# Autodesk Inventor assembly: RobotConceptTesting
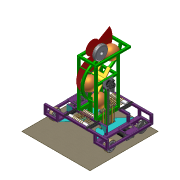
[picture p0: Inventor's stored thumbnail of the model, 180x180]
Saved by Autodesk Inventor 2012 (Build 160160000, 160)
## iProperties
Created: 2012-01-09
Part Number: RobotConceptTesting
Document SubType Name: Assembly
Designer: JesseK
Mass: 20586.5 g
Surface Area: 79739.9 cm^2
Volume: 10731.8 cm^3
Density: 1.91828 g/cm^3
Author: JesseK
## Documents named in this file (8)
- Z:\UserData\Documents\Inventor\team1885frc\Robot2012\RobotConceptTesting.iam
- Z:\UserData\Documents\Inventor\team1885frc\Robot2012\DriveTrain\DiveTrain_FullAssembly.iam
- Z:\UserData\Documents\Inventor\team1885frc\Robot2012\Concepts\Floor.ipt
- Z:\UserData\Documents\Inventor\team1885frc\Robot2012\Conveyor2\ConveyorFullAssembly.iam
- Z:\UserData\Documents\Inventor\team1885frc\Robot2012\Concepts\ShooterSketch.ipt
- Z:\UserData\Documents\Inventor\team1885frc\Robot2012\Conveyor2\Conveyor_Roller_Cross.ipt
- Z:\UserData\Documents\Inventor\team1885frc\Robot2012\Conveyor2\PitchingArmConcept.ipt
- Z:\UserData\Documents\Inventor\team1885frc\Field\Compressed ball.ipt
## Components (10 placed, 7 different names)
1. DiveTrain_FullAssembly:1 [sub-assembly] — Tangent:1, Flush:1, Flush:2, Flush:5, Mate:4, Tangent:5, Flush:8
2. Floor:1 — Tangent:1, Flush:1, Flush:2, Mate:6
3. ConveyorFullAssembly:1 [sub-assembly] — Flush:5, Mate:4, Mate:7, Mate:12, Flush:8, Tangent:6, Tangent:7
4. ShooterSketch:1 — Tangent:5, Mate:6, Mate:7, Mate:10
5. Conveyor_Roller_Cross:1 — Mate:8, Mate:9, Mate:10, Flush:7, Mate:12
6. PitchingArmConcept:1 — Mate:9, Flush:6, Flush:7, Mate:11
7. PitchingArmConcept:2 — Mate:8, Flush:6, Mate:11, Tangent:8
8. Compressed ball:1 — Tangent:6, Tangent:8
9. Compressed ball:2
10. Compressed ball:3 — Tangent:7
## Relationships (19: Mate 8, Flush 6, Tangent 5)
- Tangent:1: DiveTrain_FullAssembly:1 ↔ Floor:1
- Flush:1 (38.1 mm): DiveTrain_FullAssembly:1 ↔ Floor:1
- Flush:2 (38.1 mm): DiveTrain_FullAssembly:1 ↔ Floor:1
- Flush:5: DiveTrain_FullAssembly:1 ↔ ConveyorFullAssembly:1
- Mate:4: DiveTrain_FullAssembly:1 ↔ ConveyorFullAssembly:1
- Tangent:5: DiveTrain_FullAssembly:1 ↔ ShooterSketch:1
- Mate:6 (419.1 mm): Floor:1 ↔ ShooterSketch:1
- Mate:7: ConveyorFullAssembly:1 ↔ ShooterSketch:1
- Mate:8: Conveyor_Roller_Cross:1 ↔ PitchingArmConcept:2
- Mate:9: Conveyor_Roller_Cross:1 ↔ PitchingArmConcept:1
- Mate:10: ShooterSketch:1 ↔ Conveyor_Roller_Cross:1
- Flush:6: PitchingArmConcept:1 ↔ PitchingArmConcept:2
- Flush:7: Conveyor_Roller_Cross:1 ↔ PitchingArmConcept:1
- Mate:11: PitchingArmConcept:1 ↔ PitchingArmConcept:2
- Mate:12 (25.4 mm): ConveyorFullAssembly:1 ↔ Conveyor_Roller_Cross:1
- Flush:8 (-152.4 mm): DiveTrain_FullAssembly:1 ↔ ConveyorFullAssembly:1
- Tangent:6: ConveyorFullAssembly:1 ↔ Compressed ball:1
- Tangent:7: ConveyorFullAssembly:1 ↔ Compressed ball:3
- Tangent:8: PitchingArmConcept:2 ↔ Compressed ball:1
